# Autodesk Inventor assembly: y_carriage
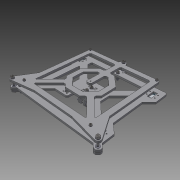
[picture p0: Inventor's stored thumbnail of the model, 180x180]
Saved by Autodesk Inventor 2014 (Build 180170000, 170)
## iProperties
Created: 2013-12-05
Part Number: y_carriage
Document SubType Name: Assembly
Designer: buben
Author: buben
## Documents named in this file (19)
- C:\Users\buben\Documents\GitHub\bacon\inventor files\assemblies\y_carriage.iam
- C:\Users\buben\Documents\GitHub\bacon\inventor files\printer parts\y_carriage.ipt
- C:\Users\buben\Documents\GitHub\bacon\inventor files\printer parts\y_carriage_belt_mount.ipt
- C:\Users\buben\Documents\GitHub\bacon\inventor files\printer parts\y_carriage_belt_mount_bed_holder.ipt
- C:\Users\buben\Documents\GitHub\bacon\inventor files\utils\washer_m4.ipt
- C:\Users\buben\Documents\Inventor\Content Center Files\R2014\en-US\ISO 4762(2)\ISO 4762 - M4 x 30ISO.ipt
- C:\Users\buben\Documents\Inventor\Content Center Files\R2014\en-US\ISO 7040\ISO 7040 - M4.ipt
- C:\Users\buben\Documents\GitHub\bacon\inventor files\printer parts\heatbed_mount.ipt
- C:\Users\buben\Documents\GitHub\bacon\inventor files\utils\washer_m5.ipt
- C:\Users\buben\Documents\GitHub\bacon\inventor files\3rd party components\linear_bearing_8\Imported Components\LU8MM\LU8MM.iam
- C:\Users\buben\Documents\GitHub\bacon\inventor files\printer parts\y_carriage_nut_holder_a.ipt
- C:\Users\buben\Documents\GitHub\bacon\inventor files\printer parts\y_carriage_nut_holder_b.ipt
- C:\Users\buben\Documents\Inventor\Content Center Files\R2014\en-US\ISO 4762(2)\ISO 4762 - M4 x 20ISO.ipt
- C:\Users\buben\Documents\Inventor\Content Center Files\R2014\en-US\ISO 4762(2)\ISO 4762 - M5 x 40ISO.ipt
- C:\Users\buben\Documents\Inventor\Content Center Files\R2014\en-US\ISO 4032(2)\ISO 4032 - M5ISO.ipt
- C:\Users\buben\Documents\Inventor\Content Center Files\R2014\en-US\ISO 4032(2)\ISO 4032 - M3ISO.ipt
- C:\Users\buben\Documents\GitHub\bacon\inventor files\utils\pcb_heatbed.ipt
- C:\Users\buben\Documents\GitHub\bacon\inventor files\utils\washer_m3.ipt
- C:\Users\buben\Documents\Inventor\Content Center Files\R2014\en-US\ISO 4762(2)\ISO 4762 - M3 x 12ISO.ipt
## Components (78 placed, 18 different names)
1. y_carriage:1 — Mate:1, Flush:1, Mate:2, Mate:9, Mate:10, Mate:11, Mate:12, Mate:13, Mate:14, Mate:15, Mate:36, Mate:37, Mate:38, Mate:51, Mate:52, Mate:53, Mate:54, Mate:55, Mate:56, Mate:57, Mate:58, Mate:59, Mate:60, Mate:61, Mate:62, Mate:63, Mate:64, Mate:65, Mate:66, Mate:67, Mate:68, Mate:69, Mate:70, Mate:71, Mate:72, Mate:73, Mate:74, Mate:75, Mate:76, Mate:77, Mate:78, Mate:79, Mate:80, Mate:82, Flush:2, Mate:84, Flush:3, Mate:86, Flush:4, Mate:90, Mate:91, Mate:92, Mate:93, Mate:94, Mate:95
2. y_carriage_belt_mount:1 — Mate:3, Mate:4, Mate:5, Mate:9, Mate:10, Mate:11, Mate:20, Mate:21, Mate:22, Mate:23
3. y_carriage_belt_mount:2 — Mate:6, Mate:7, Mate:8, Mate:24, Mate:26
4. y_carriage_belt_mount_bed_holder:1 — Mate:3, Mate:4, Mate:5, Mate:6, Mate:7, Mate:8, Mate:16, Mate:18
5. CSN 02 1702 B B 4,3:1 — Mate:12, Mate:14, Insert:2
6. CSN 02 1702 B B 4,3:2 — Mate:13, Mate:15, Insert:1
7. CSN 02 1702 B B 4,3:3 — Mate:18, Mate:19, Mate:28
8. CSN 02 1702 B B 4,3:4 — Mate:22, Mate:23, Insert:4
9. CSN 02 1702 B B 4,3:5 — Mate:24, Mate:25, Mate:32
10. CSN 02 1702 B B 4,3:6 — Mate:20, Mate:21, Insert:3
11. CSN 02 1702 B B 4,3:7 — Mate:16, Mate:17, Mate:30
12. CSN 02 1702 B B 4,3:8 — Mate:26, Mate:27, Mate:34
13. ISO 4762 M4 x 30:1 — Insert:2, Mate:19, Mate:29
14. ISO 4762 M4 x 30:2 — Insert:1, Mate:17, Mate:31
15. ISO 4762 M4 x 30:3 — Insert:3, Mate:25, Mate:33
16. ISO 4762 M4 x 30:4 — Insert:4, Mate:27, Mate:35
17. DIN EN ISO 7040 M4:1 — Mate:28, Mate:29
18. DIN EN ISO 7040 M4:2 — Mate:32, Mate:33
19. DIN EN ISO 7040 M4:3 — Mate:30, Mate:31
20. DIN EN ISO 7040 M4:4 — Mate:34, Mate:35
21. heatbed_mount:1 — Mate:36, Mate:37, Mate:38, Mate:39, Mate:40, Mate:41, Mate:42, Mate:43, Mate:44, Mate:45, Mate:46, Mate:47, Mate:48, Mate:49, Mate:50, Mate:114, Mate:115, Mate:116, Mate:125, Mate:129, Mate:133, Mate:135
22. CSN 02 1702 B B 5,3:1 — Mate:45, Mate:46
23. CSN 02 1702 B B 5,3:2 — Mate:49, Mate:50
24. CSN 02 1702 B B 5,3:3 — Mate:57, Mate:58, Mate:85, Mate:113
25. CSN 02 1702 B B 5,3:4 — Mate:55, Mate:56
26. CSN 02 1702 B B 5,3:5 — Mate:53, Mate:54
27. CSN 02 1702 B B 5,3:6 — Mate:41, Mate:42, Insert:8
28. CSN 02 1702 B B 5,3:7 — Mate:59, Mate:60, Mate:81, Mate:107
29. CSN 02 1702 B B 5,3:8 — Mate:61, Mate:62, Mate:83, Mate:110
30. CSN 02 1702 B B 5,3:9 — Mate:51, Mate:52
31. CSN 02 1702 B B 5,3:10 — Mate:47, Mate:48
32. CSN 02 1702 B B 5,3:11 — Mate:40, Mate:44, Insert:10
33. CSN 02 1702 B B 5,3:12 — Mate:39, Mate:43, Insert:9
34. LU8MM:1 [sub-assembly] — Mate:69, Mate:70, Mate:71
35. LU8MM:2 [sub-assembly] — Mate:67, Mate:68, Mate:74
36. LU8MM:3 [sub-assembly] — Mate:65, Mate:66, Mate:72
37. LU8MM:4 [sub-assembly] — Mate:63, Mate:64, Mate:73
38. CSN 02 1702 B B 4,3:9 — Mate:79, Mate:80
39. CSN 02 1702 B B 4,3:10 — Mate:77, Mate:78
40. CSN 02 1702 B B 4,3:11 — Mate:75, Mate:76
41. y_carriage_nut_holder_a:1 — Mate:83, Mate:84, Flush:3, Mate:88, Mate:108, Mate:109
42. y_carriage_nut_holder_a:2 — Mate:81, Mate:82, Flush:2, Mate:87, Mate:105, Mate:106
43. y_carriage_nut_holder_b:1 — Mate:85, Mate:86, Flush:4, Mate:89, Mate:111, Mate:112
44. CSN 02 1702 B B 4,3:12 — Mate:88, Mate:97, Mate:103
45. CSN 02 1702 B B 4,3:13 — Mate:92, Mate:93, Insert:7
46. CSN 02 1702 B B 4,3:14 — Mate:90, Mate:94, Insert:5
47. CSN 02 1702 B B 4,3:15 — Mate:91, Mate:95, Insert:6
48. CSN 02 1702 B B 4,3:16 — Mate:89, Mate:98, Mate:99
49. CSN 02 1702 B B 4,3:17 — Mate:87, Mate:96, Mate:101
50. ISO 4762 M4 x 20:1 — Insert:5, Mate:96, Mate:102
51. ISO 4762 M4 x 20:2 — Insert:6, Mate:98, Mate:100
52. ISO 4762 M4 x 20:3 — Insert:7, Mate:97, Mate:104
53. DIN EN ISO 7040 M4:5 — Mate:103, Mate:104
54. DIN EN ISO 7040 M4:6 — Mate:101, Mate:102
55. DIN EN ISO 7040 M4:7 — Mate:99, Mate:100
56. ISO 4762 M5 x 40:1 — Insert:10
57. ISO 4762 M5 x 40:2 — Insert:9
58. ISO 4762 M5 x 40:3 — Insert:8
59. ISO 4032 M5:1 — Mate:111, Mate:112, Mate:113
60. ISO 4032 M5:2 — Mate:108, Mate:109, Mate:110
61. ISO 4032 M5:3 — Mate:105, Mate:106, Mate:107
62. ISO 4032 M3:1 — Mate:139, Mate:140
63. ISO 4032 M3:2 — Mate:137, Mate:138
64. ISO 4032 M3:3 — Mate:127, Mate:128
65. ISO 4032 M3:4 — Mate:131, Mate:132
66. pcb_heatbed:1 — Mate:114, Mate:115, Mate:116, Mate:117, Mate:118, Mate:119, Mate:120, Mate:121, Mate:122, Mate:123, Mate:124
67. CSN 02 1702 B B 3,2:1 — Mate:123, Mate:124, Insert:14
68. CSN 02 1702 B B 3,2:2 — Mate:135, Mate:136, Mate:139
69. CSN 02 1702 B B 3,2:3 — Mate:133, Mate:134, Mate:137
70. CSN 02 1702 B B 3,2:4 — Mate:125, Mate:126, Mate:127
71. CSN 02 1702 B B 3,2:5 — Mate:129, Mate:130, Mate:131
72. CSN 02 1702 B B 3,2:6 — Mate:121, Mate:122, Insert:13
73. CSN 02 1702 B B 3,2:7 — Mate:119, Mate:120, Insert:12
74. CSN 02 1702 B B 3,2:8 — Mate:117, Mate:118, Insert:11
75. ISO 4762 M3 x 12:1 — Insert:14, Mate:136, Mate:140
76. ISO 4762 M3 x 12:2 — Insert:13, Mate:134, Mate:138
77. ISO 4762 M3 x 12:3 — Insert:11, Mate:126, Mate:128
78. ISO 4762 M3 x 12:4 — Insert:12, Mate:130, Mate:132
## Relationships (158: Mate 140, Insert 14, Flush 4)
- Mate:1: y_carriage:1
- Flush:1: y_carriage:1
- Mate:2: y_carriage:1
- Mate:3: y_carriage_belt_mount:1 ↔ y_carriage_belt_mount_bed_holder:1
- Mate:4: y_carriage_belt_mount:1 ↔ y_carriage_belt_mount_bed_holder:1
- Mate:5: y_carriage_belt_mount:1 ↔ y_carriage_belt_mount_bed_holder:1
- Mate:6: y_carriage_belt_mount:2 ↔ y_carriage_belt_mount_bed_holder:1
- Mate:7: y_carriage_belt_mount:2 ↔ y_carriage_belt_mount_bed_holder:1
- Mate:8: y_carriage_belt_mount:2 ↔ y_carriage_belt_mount_bed_holder:1
- Mate:9: y_carriage:1 ↔ y_carriage_belt_mount:1
- Mate:10: y_carriage:1 ↔ y_carriage_belt_mount:1
- Mate:11: y_carriage:1 ↔ y_carriage_belt_mount:1
- Mate:12: y_carriage:1 ↔ CSN 02 1702 B B 4,3:1
- Mate:13: y_carriage:1 ↔ CSN 02 1702 B B 4,3:2
- Mate:14: y_carriage:1 ↔ CSN 02 1702 B B 4,3:1
- Mate:15: y_carriage:1 ↔ CSN 02 1702 B B 4,3:2
- Insert:1: CSN 02 1702 B B 4,3:2 ↔ ISO 4762 M4 x 30:2
- Insert:2: CSN 02 1702 B B 4,3:1 ↔ ISO 4762 M4 x 30:1
- Mate:16: y_carriage_belt_mount_bed_holder:1 ↔ CSN 02 1702 B B 4,3:7
- Mate:17: CSN 02 1702 B B 4,3:7 ↔ ISO 4762 M4 x 30:2
- Mate:18: y_carriage_belt_mount_bed_holder:1 ↔ CSN 02 1702 B B 4,3:3
- Mate:19: CSN 02 1702 B B 4,3:3 ↔ ISO 4762 M4 x 30:1
- Mate:20: y_carriage_belt_mount:1 ↔ CSN 02 1702 B B 4,3:6
- Mate:21: y_carriage_belt_mount:1 ↔ CSN 02 1702 B B 4,3:6
- Mate:22: y_carriage_belt_mount:1 ↔ CSN 02 1702 B B 4,3:4
- Mate:23: y_carriage_belt_mount:1 ↔ CSN 02 1702 B B 4,3:4
- Insert:3: CSN 02 1702 B B 4,3:6 ↔ ISO 4762 M4 x 30:3
- Insert:4: CSN 02 1702 B B 4,3:4 ↔ ISO 4762 M4 x 30:4
- Mate:24: y_carriage_belt_mount:2 ↔ CSN 02 1702 B B 4,3:5
- Mate:25: CSN 02 1702 B B 4,3:5 ↔ ISO 4762 M4 x 30:3
- Mate:26: y_carriage_belt_mount:2 ↔ CSN 02 1702 B B 4,3:8
- Mate:27: CSN 02 1702 B B 4,3:8 ↔ ISO 4762 M4 x 30:4
- Mate:28: CSN 02 1702 B B 4,3:3 ↔ DIN EN ISO 7040 M4:1
- Mate:29: ISO 4762 M4 x 30:1 ↔ DIN EN ISO 7040 M4:1
- Mate:30: CSN 02 1702 B B 4,3:7 ↔ DIN EN ISO 7040 M4:3
- Mate:31: ISO 4762 M4 x 30:2 ↔ DIN EN ISO 7040 M4:3
- Mate:32: CSN 02 1702 B B 4,3:5 ↔ DIN EN ISO 7040 M4:2
- Mate:33: ISO 4762 M4 x 30:3 ↔ DIN EN ISO 7040 M4:2
- Mate:34: CSN 02 1702 B B 4,3:8 ↔ DIN EN ISO 7040 M4:4
- Mate:35: ISO 4762 M4 x 30:4 ↔ DIN EN ISO 7040 M4:4
- Mate:36 (15 mm): y_carriage:1 ↔ heatbed_mount:1
- Mate:37: y_carriage:1 ↔ heatbed_mount:1
- Mate:38: y_carriage:1 ↔ heatbed_mount:1
- Mate:39: heatbed_mount:1 ↔ CSN 02 1702 B B 5,3:12
- Mate:40: heatbed_mount:1 ↔ CSN 02 1702 B B 5,3:11
- Mate:41: heatbed_mount:1 ↔ CSN 02 1702 B B 5,3:6
- Mate:42: heatbed_mount:1 ↔ CSN 02 1702 B B 5,3:6
- Mate:43: heatbed_mount:1 ↔ CSN 02 1702 B B 5,3:12
- Mate:44: heatbed_mount:1 ↔ CSN 02 1702 B B 5,3:11
- Mate:45: heatbed_mount:1 ↔ CSN 02 1702 B B 5,3:1
- Mate:46: heatbed_mount:1 ↔ CSN 02 1702 B B 5,3:1
- Mate:47: heatbed_mount:1 ↔ CSN 02 1702 B B 5,3:10
- Mate:48: heatbed_mount:1 ↔ CSN 02 1702 B B 5,3:10
- Mate:49: heatbed_mount:1 ↔ CSN 02 1702 B B 5,3:2
- Mate:50: heatbed_mount:1 ↔ CSN 02 1702 B B 5,3:2
- Mate:51: y_carriage:1 ↔ CSN 02 1702 B B 5,3:9
- Mate:52: y_carriage:1 ↔ CSN 02 1702 B B 5,3:9
- Mate:53: y_carriage:1 ↔ CSN 02 1702 B B 5,3:5
- Mate:54: y_carriage:1 ↔ CSN 02 1702 B B 5,3:5
- Mate:55: y_carriage:1 ↔ CSN 02 1702 B B 5,3:4
- Mate:56: y_carriage:1 ↔ CSN 02 1702 B B 5,3:4
- Mate:57: y_carriage:1 ↔ CSN 02 1702 B B 5,3:3
- Mate:58: y_carriage:1 ↔ CSN 02 1702 B B 5,3:3
- Mate:59: y_carriage:1 ↔ CSN 02 1702 B B 5,3:7
- Mate:60: y_carriage:1 ↔ CSN 02 1702 B B 5,3:7
- Mate:61: y_carriage:1 ↔ CSN 02 1702 B B 5,3:8
- Mate:62: y_carriage:1 ↔ CSN 02 1702 B B 5,3:8
- Mate:63 (7.5 mm): y_carriage:1 ↔ LU8MM:4
- Mate:64 (7.5 mm): y_carriage:1 ↔ LU8MM:4
- Mate:65 (7.5 mm): y_carriage:1 ↔ LU8MM:3
- Mate:66 (7.5 mm): y_carriage:1 ↔ LU8MM:3
- Mate:67 (7.5 mm): y_carriage:1 ↔ LU8MM:2
- Mate:68 (7.5 mm): y_carriage:1 ↔ LU8MM:2
- Mate:69 (7.5 mm): y_carriage:1 ↔ LU8MM:1
- Mate:70 (7.5 mm): y_carriage:1 ↔ LU8MM:1
- Mate:71 (0.5 mm): y_carriage:1 ↔ LU8MM:1
- Mate:72 (0.5 mm): y_carriage:1 ↔ LU8MM:3
- Mate:73 (0.5 mm): y_carriage:1 ↔ LU8MM:4
- Mate:74 (0.5 mm): y_carriage:1 ↔ LU8MM:2
- Mate:75: y_carriage:1 ↔ CSN 02 1702 B B 4,3:11
- Mate:76: y_carriage:1 ↔ CSN 02 1702 B B 4,3:11
- Mate:77: y_carriage:1 ↔ CSN 02 1702 B B 4,3:10
- Mate:78: y_carriage:1 ↔ CSN 02 1702 B B 4,3:10
- Mate:79: y_carriage:1 ↔ CSN 02 1702 B B 4,3:9
- Mate:80: y_carriage:1 ↔ CSN 02 1702 B B 4,3:9
- Mate:81: CSN 02 1702 B B 5,3:7 ↔ y_carriage_nut_holder_a:2
- Mate:82: y_carriage:1 ↔ y_carriage_nut_holder_a:2
- Flush:2: y_carriage:1 ↔ y_carriage_nut_holder_a:2
- Mate:83: CSN 02 1702 B B 5,3:8 ↔ y_carriage_nut_holder_a:1
- Mate:84: y_carriage:1 ↔ y_carriage_nut_holder_a:1
- Flush:3: y_carriage:1 ↔ y_carriage_nut_holder_a:1
- Mate:85: CSN 02 1702 B B 5,3:3 ↔ y_carriage_nut_holder_b:1
- Mate:86: y_carriage:1 ↔ y_carriage_nut_holder_b:1
- Flush:4: y_carriage:1 ↔ y_carriage_nut_holder_b:1
- Mate:87: y_carriage_nut_holder_a:2 ↔ CSN 02 1702 B B 4,3:17
- Mate:88: y_carriage_nut_holder_a:1 ↔ CSN 02 1702 B B 4,3:12
- Mate:89: y_carriage_nut_holder_b:1 ↔ CSN 02 1702 B B 4,3:16
- Mate:90: y_carriage:1 ↔ CSN 02 1702 B B 4,3:14
- Mate:91: y_carriage:1 ↔ CSN 02 1702 B B 4,3:15
- Mate:92: y_carriage:1 ↔ CSN 02 1702 B B 4,3:13
- Mate:93: y_carriage:1 ↔ CSN 02 1702 B B 4,3:13
- Mate:94: y_carriage:1 ↔ CSN 02 1702 B B 4,3:14
- Mate:95: y_carriage:1 ↔ CSN 02 1702 B B 4,3:15
- Insert:5: CSN 02 1702 B B 4,3:14 ↔ ISO 4762 M4 x 20:1
- Insert:6: CSN 02 1702 B B 4,3:15 ↔ ISO 4762 M4 x 20:2
- Insert:7: CSN 02 1702 B B 4,3:13 ↔ ISO 4762 M4 x 20:3
- Mate:96: CSN 02 1702 B B 4,3:17 ↔ ISO 4762 M4 x 20:1
- Mate:97: CSN 02 1702 B B 4,3:12 ↔ ISO 4762 M4 x 20:3
- Mate:98: CSN 02 1702 B B 4,3:16 ↔ ISO 4762 M4 x 20:2
- Mate:99: CSN 02 1702 B B 4,3:16 ↔ DIN EN ISO 7040 M4:7
- Mate:100: ISO 4762 M4 x 20:2 ↔ DIN EN ISO 7040 M4:7
- Mate:101: CSN 02 1702 B B 4,3:17 ↔ DIN EN ISO 7040 M4:6
- Mate:102: ISO 4762 M4 x 20:1 ↔ DIN EN ISO 7040 M4:6
- Mate:103: CSN 02 1702 B B 4,3:12 ↔ DIN EN ISO 7040 M4:5
- Mate:104: ISO 4762 M4 x 20:3 ↔ DIN EN ISO 7040 M4:5
- Insert:8: CSN 02 1702 B B 5,3:6 ↔ ISO 4762 M5 x 40:3
- Insert:9: CSN 02 1702 B B 5,3:12 ↔ ISO 4762 M5 x 40:2
- Insert:10: CSN 02 1702 B B 5,3:11 ↔ ISO 4762 M5 x 40:1
- Mate:105: y_carriage_nut_holder_a:2 ↔ ISO 4032 M5:3
- Mate:106: y_carriage_nut_holder_a:2 ↔ ISO 4032 M5:3
- Mate:107: CSN 02 1702 B B 5,3:7 ↔ ISO 4032 M5:3
- Mate:108: y_carriage_nut_holder_a:1 ↔ ISO 4032 M5:2
- Mate:109: y_carriage_nut_holder_a:1 ↔ ISO 4032 M5:2
- Mate:110: CSN 02 1702 B B 5,3:8 ↔ ISO 4032 M5:2
- Mate:111: y_carriage_nut_holder_b:1 ↔ ISO 4032 M5:1
- Mate:112: y_carriage_nut_holder_b:1 ↔ ISO 4032 M5:1
- Mate:113: CSN 02 1702 B B 5,3:3 ↔ ISO 4032 M5:1
- Mate:114: heatbed_mount:1 ↔ pcb_heatbed:1
- Mate:115: heatbed_mount:1 ↔ pcb_heatbed:1
- Mate:116: heatbed_mount:1 ↔ pcb_heatbed:1
- Mate:117: pcb_heatbed:1 ↔ CSN 02 1702 B B 3,2:8
- Mate:118: pcb_heatbed:1 ↔ CSN 02 1702 B B 3,2:8
- Mate:119: pcb_heatbed:1 ↔ CSN 02 1702 B B 3,2:7
- Mate:120: pcb_heatbed:1 ↔ CSN 02 1702 B B 3,2:7
- Mate:121: pcb_heatbed:1 ↔ CSN 02 1702 B B 3,2:6
- Mate:122: pcb_heatbed:1 ↔ CSN 02 1702 B B 3,2:6
- Mate:123: pcb_heatbed:1 ↔ CSN 02 1702 B B 3,2:1
- Mate:124: pcb_heatbed:1 ↔ CSN 02 1702 B B 3,2:1
- Insert:11: CSN 02 1702 B B 3,2:8 ↔ ISO 4762 M3 x 12:3
- Mate:125: heatbed_mount:1 ↔ CSN 02 1702 B B 3,2:4
- Mate:126: CSN 02 1702 B B 3,2:4 ↔ ISO 4762 M3 x 12:3
- Mate:127: ISO 4032 M3:3 ↔ CSN 02 1702 B B 3,2:4
- Mate:128: ISO 4032 M3:3 ↔ ISO 4762 M3 x 12:3
- Insert:12: CSN 02 1702 B B 3,2:7 ↔ ISO 4762 M3 x 12:4
- Mate:129: heatbed_mount:1 ↔ CSN 02 1702 B B 3,2:5
- Mate:130: CSN 02 1702 B B 3,2:5 ↔ ISO 4762 M3 x 12:4
- Mate:131: ISO 4032 M3:4 ↔ CSN 02 1702 B B 3,2:5
- Mate:132: ISO 4032 M3:4 ↔ ISO 4762 M3 x 12:4
- Insert:13: CSN 02 1702 B B 3,2:6 ↔ ISO 4762 M3 x 12:2
- Insert:14: CSN 02 1702 B B 3,2:1 ↔ ISO 4762 M3 x 12:1
- Mate:133: heatbed_mount:1 ↔ CSN 02 1702 B B 3,2:3
- Mate:134: CSN 02 1702 B B 3,2:3 ↔ ISO 4762 M3 x 12:2
- Mate:135: heatbed_mount:1 ↔ CSN 02 1702 B B 3,2:2
- Mate:136: CSN 02 1702 B B 3,2:2 ↔ ISO 4762 M3 x 12:1
- Mate:137: ISO 4032 M3:2 ↔ CSN 02 1702 B B 3,2:3
- Mate:138: ISO 4032 M3:2 ↔ ISO 4762 M3 x 12:2
- Mate:139: ISO 4032 M3:1 ↔ CSN 02 1702 B B 3,2:2
- Mate:140: ISO 4032 M3:1 ↔ ISO 4762 M3 x 12:1
